# Autodesk Inventor assembly: 111_onering_soro
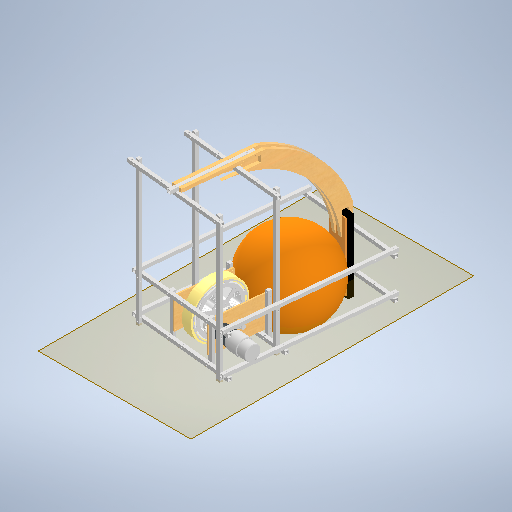
[picture p0: Inventor's stored thumbnail of the model, 512x512]
Saved by Autodesk Inventor 2025.1 (Build 291241000, 241)
## iProperties
Created: 2024-10-08
Part Number: 111_onering_soro
Document SubType Name: Assembly
Designer: yuki0520
Author: yuki0520
## Documents named in this file (5)
- C:\Users\yuki0520\OneDrive\ドキュメント\Inventor\2025_nhk\tanaka\nageru\onering\111_onering_soro.iam
- C:\Users\yuki0520\OneDrive\ドキュメント\Inventor\2025_nhk\tanaka\object\ball.ipt
- C:\Users\yuki0520\OneDrive\ドキュメント\Inventor\2025_nhk\tanaka\nageru\pakuriz\TH22_soroban_sn.ipt
- C:\Users\yuki0520\OneDrive\ドキュメント\Inventor\2025_nhk\tanaka\nageru\onering\onering_tire_set.iam
- C:\Users\yuki0520\OneDrive\ドキュメント\Inventor\2025_nhk\tanaka\nageru\onering\rail_test_90.ipt
## Components (5 placed, 4 different names)
1. ball:1 — 正接:1
2. TH22_soroban_sn:1 — 挿入:48, 挿入:49
3. onering_tire_set:1 [sub-assembly] — 挿入:48, 挿入:49, 正接:1, 挿入:50, 挿入:51, 挿入:52, 挿入:53, メイト:1
4. rail_test_90:1 — 挿入:52, 挿入:53
5. rail_test_90:2 — 挿入:50, 挿入:51
## Relationships (8: Insert 6, Tangent 1, Mate 1)
- 挿入:48 [Insert]: TH22_soroban_sn:1 ↔ onering_tire_set:1
- 挿入:49 [Insert]: TH22_soroban_sn:1 ↔ onering_tire_set:1
- 正接:1 [Tangent]: ball:1 ↔ onering_tire_set:1
- 挿入:50 [Insert]: onering_tire_set:1 ↔ rail_test_90:2
- 挿入:51 [Insert]: onering_tire_set:1 ↔ rail_test_90:2
- 挿入:52 [Insert]: onering_tire_set:1 ↔ rail_test_90:1
- 挿入:53 [Insert]: onering_tire_set:1 ↔ rail_test_90:1
- メイト:1 [Mate]: onering_tire_set:1
